# Autodesk Inventor assembly: Thermal cover assembly
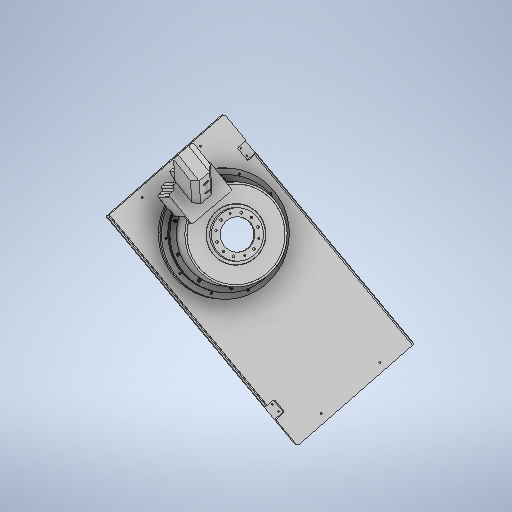
[picture p0: Inventor's stored thumbnail of the model, 512x512]
Saved by Autodesk Inventor 2025.2 (Build 292293000, 293)
## iProperties
Created: 2025-07-25
Part Number: Thermal cover assembly
Document SubType Name: Assembly
Designer: mateo
Author: mateo
## Documents named in this file (14)
- C:\GitHub\In-situ-monitoring-of-powder-bed-fusion-additive-manufacturing\system_development\Adamant\v0.1\hardware design\Thermal cover assembly.iam
- C:\GitHub\In-situ-monitoring-of-powder-bed-fusion-additive-manufacturing\system_development\Adamant\v0.1\hardware design\Cover (Thermal Camera).ipt
- C:\GitHub\In-situ-monitoring-of-powder-bed-fusion-additive-manufacturing\system_development\Adamant\v0.1\hardware design\300mm Housing 1.ipt
- C:\GitHub\In-situ-monitoring-of-powder-bed-fusion-additive-manufacturing\system_development\Adamant\v0.1\hardware design\300mm housing 2 Camera.ipt
- C:\GitHub\In-situ-monitoring-of-powder-bed-fusion-additive-manufacturing\system_development\Adamant\v0.1\hardware design\Cylinder Segment  Camera only v0.2.ipt
- C:\GitHub\In-situ-monitoring-of-powder-bed-fusion-additive-manufacturing\system_development\Adamant\v0.1\hardware design\Cylinder Slidey Bit Housing Camera only v0.2.ipt
- C:\GitHub\In-situ-monitoring-of-powder-bed-fusion-additive-manufacturing\system_development\Adamant\v0.1\hardware design\Cylinder Segment Holder.ipt
- C:\GitHub\In-situ-monitoring-of-powder-bed-fusion-additive-manufacturing\system_development\Adamant\v0.1\hardware design\Cylinder Segment Camera Only\C .Replace - 10.ipt
- C:\GitHub\In-situ-monitoring-of-powder-bed-fusion-additive-manufacturing\system_development\Adamant\v0.1\hardware design\Cylinder Segment Camera Only.ipt
- C:\GitHub\In-situ-monitoring-of-powder-bed-fusion-additive-manufacturing\system_development\Adamant\v0.1\hardware design\Thermal Camera Bracket.ipt
- C:\GitHub\In-situ-monitoring-of-powder-bed-fusion-additive-manufacturing\system_development\Adamant\v0.1\hardware design\C .Replace - Face.ipt
- C:\GitHub\In-situ-monitoring-of-powder-bed-fusion-additive-manufacturing\system_development\Adamant\v0.1\hardware design\Thermal Cover.ipt
- C:\GitHub\In-situ-monitoring-of-powder-bed-fusion-additive-manufacturing\system_development\Adamant\v0.1\hardware design\Welding Glass.ipt
- C:\GitHub\In-situ-monitoring-of-powder-bed-fusion-additive-manufacturing\system_development\Damascus\v0.2\Hardware\Xi 410 Camera.iam
## Components (12 placed, 12 different names)
1. Cover (Thermal Camera):1 — Insert:1, Insert:2, Insert:3
2. 300mm Housing 1:1 — Insert:1, Insert:2, Insert:3, Insert:4, Insert:5
3. 300mm housing 2 Camera:1 — Insert:4, Insert:5, Insert:6, Insert:7
4. Cylinder Segment  Camera only v0.2:1 — Insert:6, Insert:7, Insert:8, Insert:9, Insert:10, Insert:11, Mate:1
5. Cylinder Slidey Bit Housing Camera only v0.2:1 — Insert:8, Insert:9, Insert:14, Insert:15, Mate:2
6. Cylinder Segment Holder:1 — Insert:10, Insert:11, Insert:12, Insert:13
7. C .Replace - 10:1 — Insert:12
8. Thermal Camera Bracket:1 — Insert:14, Insert:15
9. C .Replace - Face:2 — Insert:13
10. Thermal Cover:1 — Mate:1
11. Welding Glass:1 — Mate:2
12. Xi 410 Camera:1 [sub-assembly]
## Relationships (17: Insert 15, Mate 2)
- Insert:1: Cover (Thermal Camera):1 ↔ 300mm Housing 1:1
- Insert:2: Cover (Thermal Camera):1 ↔ 300mm Housing 1:1
- Insert:3: Cover (Thermal Camera):1 ↔ 300mm Housing 1:1
- Insert:4: 300mm Housing 1:1 ↔ 300mm housing 2 Camera:1
- Insert:5: 300mm Housing 1:1 ↔ 300mm housing 2 Camera:1
- Insert:6 (10 mm): 300mm housing 2 Camera:1 ↔ Cylinder Segment  Camera only v0.2:1
- Insert:7 (10 mm): 300mm housing 2 Camera:1 ↔ Cylinder Segment  Camera only v0.2:1
- Insert:8: Cylinder Segment  Camera only v0.2:1 ↔ Cylinder Slidey Bit Housing Camera only v0.2:1
- Insert:9: Cylinder Segment  Camera only v0.2:1 ↔ Cylinder Slidey Bit Housing Camera only v0.2:1
- Insert:10: Cylinder Segment  Camera only v0.2:1 ↔ Cylinder Segment Holder:1
- Insert:11: Cylinder Segment  Camera only v0.2:1 ↔ Cylinder Segment Holder:1
- Insert:12: Cylinder Segment Holder:1 ↔ C .Replace - 10:1
- Insert:13: Cylinder Segment Holder:1 ↔ C .Replace - Face:2
- Insert:14: Cylinder Slidey Bit Housing Camera only v0.2:1 ↔ Thermal Camera Bracket:1
- Insert:15: Cylinder Slidey Bit Housing Camera only v0.2:1 ↔ Thermal Camera Bracket:1
- Mate:1: Cylinder Segment  Camera only v0.2:1 ↔ Thermal Cover:1
- Mate:2: Cylinder Slidey Bit Housing Camera only v0.2:1 ↔ Welding Glass:1
